# Autodesk Inventor assembly: Magisterka
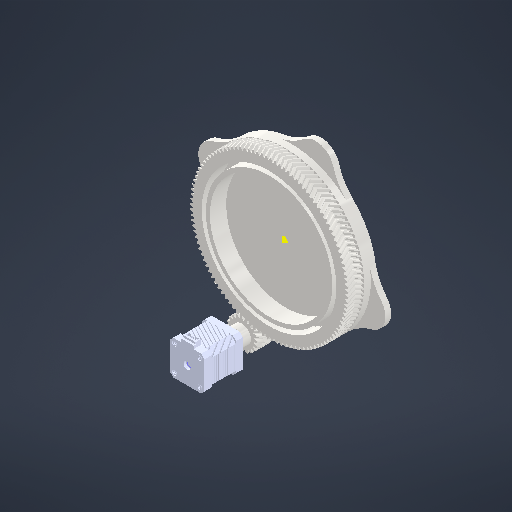
[picture p0: Inventor's stored thumbnail of the model, 512x512]
Saved by Autodesk Inventor 2026.1 (Build 301233020, 233B)
## iProperties
Created: 2025-11-16
Part Number: Magisterka
Document SubType Name: Assembly
Designer: obiwa
Author: obiwa
## Documents named in this file (3)
- C:\Users\obiwa\Desktop\Studia\Magisterka\Master-Thesis\Model\Magisterka.iam
- C:\Users\obiwa\Desktop\Studia\Magisterka\Master-Thesis\Model\Magisterka\Design Accelerator\Przekładnie walcowe1.iam
- C:\Users\obiwa\Desktop\Studia\Magisterka\Master-Thesis\Model\Magisterka\stepper-motor-nema-17-solidworks-1.snapshot.1\Stepper\Stepper\Stepper.ipt
## Components (2 placed, 2 different names)
1. Przekładnie walcowe:1 [sub-assembly] — Zestawiające:1, Zestawiające:2, Kątowe:2
2. Stepper:1 — Zestawiające:1, Zestawiające:2
## Relationships (3: Mate 2, Angle 1)
- Zestawiające:1 [Mate]: Przekładnie walcowe:1 ↔ Stepper:1
- Zestawiające:2 [Mate] (2 mm): Przekładnie walcowe:1 ↔ Stepper:1
- Kątowe:2 [Angle] (0 deg): Przekładnie walcowe:1
